# Autodesk Inventor assembly: topplate Assy
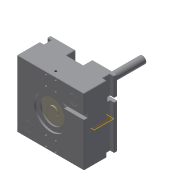
[picture p0: Inventor's stored thumbnail of the model, 180x180]
Saved by Autodesk Inventor 2022 (Build 260148000, 148)
## iProperties
Shininess: 64.0
Length Units: 11272
Angle Units: 11279
Time Units: 11290
Mass Units: 11286
Length Display Precision: 3
Angle Display Precision: 2
Compacted: True
Part Number: topplate Assy
Document SubType Name: Assembly
Created: 2003-04-07
Designer: demo
Density: 0.0
Volumn: 0.0
Area: 0.0
PropertySet Name: Model Information
Control State: 0
Master: False
Checked Out: False
Author: demo
## Documents named in this file (5)
- C:\Autodesk Inventor 2022 Advanced Assembly Modeling Practice Files\Mold Assembly\topplate Assy.iam
- C:\Autodesk Inventor 2022 Advanced Assembly Modeling Practice Files\Mold Assembly\topplate.ipt
- C:\Autodesk Inventor 2022 Advanced Assembly Modeling Practice Files\Mold Assembly\top plate washer.ipt
- C:\Autodesk Inventor 2022 Advanced Assembly Modeling Practice Files\Mold Assembly\plunger.ipt
- C:\Autodesk Inventor 2022 Advanced Assembly Modeling Practice Files\Mold Assembly\Pin1-P1.ipt
## Components (5 placed, 4 different names)
1. topplate:1 — Flush:1, Flush:2, Flush:3, Insert:1, Insert:2
2. top plate washer:1 — Flush:1
3. plunger:1 — Flush:3
4. Pin1-P1:1 — Insert:1
5. Pin1-P1:2 — Insert:2
## Relationships (5: Flush 3, Insert 2)
- Flush:1: topplate:1 ↔ top plate washer:1
- Flush:2: topplate:1
- Flush:3: topplate:1 ↔ plunger:1
- Insert:1: topplate:1 ↔ Pin1-P1:1
- Insert:2: topplate:1 ↔ Pin1-P1:2
